# Autodesk Inventor assembly: boom
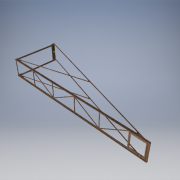
[picture p0: Inventor's stored thumbnail of the model, 180x180]
Saved by Autodesk Inventor 2018.3 (Build 223284000, 284)
## iProperties
Created: 2018-05-24
Part Number: boom
Document SubType Name: Assembly
Designer: mzhang
Mass: 13.1465 g
Surface Area: 476.751 cm^2
Volume: 23.9027 cm^3
Density: 0.55 g/cm^3
Author: mzhang
## Documents named in this file (10)
- C:\Users\mzhang\3D Objects\boom.iam
- C:\Users\mzhang\3D Objects\side.ipt
- C:\Users\mzhang\3D Objects\bottom.ipt
- C:\Users\mzhang\3D Objects\back.ipt
- C:\Users\mzhang\3D Objects\boom\AIP\FEA\citrhuacg.fins
- C:\Users\mzhang\3D Objects\boom\AIP\FEA\citrhuacg.fsat
- C:\Users\mzhang\3D Objects\boom\AIP\FEA\citrhuacg.ftes
- C:\Users\mzhang\3D Objects\boom\AIP\FEA\citrhuacg.fwiz
- C:\Users\mzhang\3D Objects\boom\AIP\FEA\citrhuaqo.fmsh
- C:\Users\mzhang\3D Objects\boom\AIP\FEA\citrhuaqp.fres
## Components (4 placed, 3 different names)
1. side:1 — Mate:1, Mate:2, Mate:3, Mate:4, Mate:7, Mate:8
2. bottom:1 — Mate:1, Mate:2, Mate:3, Mate:4, Mate:5, Flush:1, Mate:6
3. side:2 — Mate:5, Flush:1, Mate:6, Flush:2
4. back:1 — Flush:2, Mate:7, Mate:8
## Relationships (10: Mate 8, Flush 2)
- Mate:1: side:1 ↔ bottom:1
- Mate:2: side:1 ↔ bottom:1
- Mate:3: side:1 ↔ bottom:1
- Mate:4: side:1 ↔ bottom:1
- Mate:5: bottom:1 ↔ side:2
- Flush:1: bottom:1 ↔ side:2
- Mate:6: bottom:1 ↔ side:2
- Flush:2: side:2 ↔ back:1
- Mate:7: side:1 ↔ back:1
- Mate:8: side:1 ↔ back:1
## Named parameters: sa_0 = 3750, sa_1 = 3e-12, sa_2 = -3750, sa_3 = -2e-13
note: some values were not read from the file. Shown as the stored number, unit unknown: "sa_0", "sa_1", "sa_2", "sa_3".
